# Autodesk Inventor assembly: 部件1
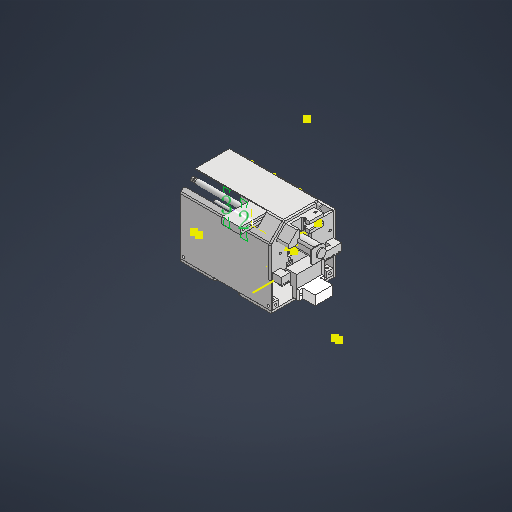
[picture p0: Inventor's stored thumbnail of the model, 512x512]
Saved by Autodesk Inventor 2025 (Build 290162000, 162)
## iProperties
Created: 2025-11-30
Part Number: 部件1
Document SubType Name: Assembly
Designer: XH
Author: XH
## Documents named in this file (41)
- C:\1A_Engineering_files\braille-printer-v2\3D文件\部件1.iam
- C:\1A_Engineering_files\braille-printer-v2\3D文件\便签.ipt
- C:\1A_Engineering_files\braille-printer-v2\3D文件\针头主体.iam
- C:\1A_Engineering_files\braille-printer-v2\3D文件\钢轴.ipt
- C:\1A_Engineering_files\braille-printer-v2\3D文件\阻挡X轴.ipt
- C:\Users\XH\Documents\Inventor\Content Center Files\R2025\zh-CN\AS 1420\AS 1420 - 1973 - M3 x 8.ipt
- C:\1A_Engineering_files\braille-printer-v2\3D文件\皮带.ipt
- C:\1A_Engineering_files\braille-printer-v2\3D文件\新配件\棍.ipt
- C:\1A_Engineering_files\braille-printer-v2\3D文件\电机.ipt
- C:\1A_Engineering_files\braille-printer-v2\3D文件\新配件\单轴.ipt
- C:\1A_Engineering_files\braille-printer-v2\3D文件\新配件\针头.iam
- C:\1A_Engineering_files\braille-printer-v2\3D文件\新配件\短轴3.ipt
- C:\1A_Engineering_files\braille-printer-v2\3D文件\新配件\连接件.ipt
- C:\1A_Engineering_files\braille-printer-v2\3D文件\阻挡X轴1.ipt
- C:\1A_Engineering_files\braille-printer-v2\3D文件\新配件\联轴器.ipt
- C:\1A_Engineering_files\braille-printer-v2\3D文件\新配件\外壳.ipt
- C:\1A_Engineering_files\braille-printer-v2\3D文件\新配件\大外壳.ipt
- C:\1A_Engineering_files\braille-printer-v2\3D文件\8D0A9F84C0C62D41F58A2185E0A23325.ipt
- C:\1A_Engineering_files\braille-printer-v2\3D文件\电机转接板.ipt
- C:\1A_Engineering_files\braille-printer-v2\3D文件\新配件\连接件电机.ipt
- C:\1A_Engineering_files\braille-printer-v2\3D文件\新配件\底板.ipt
- C:\1A_Engineering_files\braille-printer-v2\3D文件\新配件\底板2.ipt
- C:\1A_Engineering_files\braille-printer-v2\3D文件\新配件\8X.ipt
- C:\1A_Engineering_files\braille-printer-v2\3D文件\电池.ipt
- C:\1A_Engineering_files\braille-printer-v2\3D文件\ESP32.ipt
- C:\1A_Engineering_files\braille-printer-v2\3D文件\轴承3.7.3.ipt
- C:\1A_Engineering_files\braille-printer-v2\3D文件\入纸卡件.ipt
- C:\1A_Engineering_files\braille-printer-v2\3D文件\obj_2_1.齿条.STEP.ipt
- C:\1A_Engineering_files\braille-printer-v2\3D文件\obj_1_齿轮.STEP.ipt
- C:\1A_Engineering_files\braille-printer-v2\3D文件\Y轴杠轴.ipt
- C:\1A_Engineering_files\braille-printer-v2\3D文件\obj_3_外壳.STL.ipt
- C:\1A_Engineering_files\braille-printer-v2\3D文件\新配件\obj_2_1.齿条.STEP.ipt
- C:\1A_Engineering_files\braille-printer-v2\3D文件\obj_3_外1壳.STL.ipt
- C:\1A_Engineering_files\braille-printer-v2\3D文件\外宽挤压.ipt
- C:\1A_Engineering_files\braille-printer-v2\3D文件\小短轴.ipt
- C:\1A_Engineering_files\braille-printer-v2\3D文件\前轴固定.ipt
- C:\1A_Engineering_files\braille-printer-v2\3D文件\轴套.ipt
- C:\1A_Engineering_files\braille-printer-v2\3D文件\打印伸缩轴.ipt
- C:\1A_Engineering_files\braille-printer-v2\3D文件\铜套.ipt
- C:\1A_Engineering_files\braille-printer-v2\3D文件\新配件\滚纸.ipt
- C:\1A_Engineering_files\braille-printer-v2\3D文件\Z轴.ipt
## Components (66 placed, 39 different names)
1. 便签:1
2. 针头主体:1 [sub-assembly] — 配合:5, 配合:34, 表面齐平:19, 配合:198, 配合:199, 配合:200
3. 钢轴:2 — 配合:5, 表面齐平:14, 配合:83
4. 钢轴:3 — 配合:34, 表面齐平:14, 配合:75, 配合:76, 配合:82
5. AS 1420 - 公制 M3 x 8:1 — 配合:79, 配合:80
6. AS 1420 - 公制 M3 x 8:2 — 配合:77, 配合:78
7. 皮带:1
8. 棍:1 — 表面齐平:18, 配合:72
9. 棍:3 — 表面齐平:16, 配合:70
10. 棍:5 — 表面齐平:17, 配合:71
11. 电机:1 — 配合:73
12. 棍:6 — 表面齐平:18, 配合:68
13. 棍:7 — 表面齐平:16, 配合:69
14. 棍:8 — 表面齐平:17, 配合:67
15. 单轴:1
16. 针头:1 [sub-assembly] — 表面齐平:19, 配合:193, 配合:194, 配合:195, 配合:196, 配合:198, 配合:199, 配合:200
17. 短轴3:1 — 配合:67, 配合:68, 配合:69, 配合:201, 配合:204, 配合:211, 配合:214, 配合:288
18. 短轴3:2 — 配合:70, 配合:71, 配合:72, 配合:73, 配合:103, 配合:203, 表面齐平:29, 配合:212, 配合:289
19. 阻挡X轴:2 — 配合:75, 配合:76, 配合:77, 配合:78, 配合:79, 配合:80, 配合:100, 表面齐平:24, 表面齐平:25, 配合:210, 配合:213, 表面齐平:40, 配合:266, 配合:275, 配合:277, 配合:280
20. 连接件:1 — 配合:100, 配合:210, 配合:212, 配合:213, 配合:214
21. 阻挡X轴1:1 — 配合:82, 配合:83, 配合:104, 配合:105, 配合:123, 配合:221, 表面齐平:30, 表面齐平:31, 表面齐平:32, 配合:233, 表面齐平:33, 配合:234, 配合:278, 配合:293
22. 联轴器:1 — 配合:103
23. 外壳:1 — 配合:104
24. 大外壳:1 — 配合:105, 表面齐平:27, 配合:282, 配合:283, 配合:284
25. 电机转接板:1
26. 连接件电机:1 — 配合:123
27. 底板:1 — 表面齐平:24, 表面齐平:27, 配合:197, 表面齐平:28, 表面齐平:40, 配合:264, 表面齐平:43, 配合:275, 配合:281, 表面齐平:44, 配合:285, 配合:287
28. 底板2:1 — 表面齐平:25, 配合:232, 配合:234, 配合:265, 表面齐平:43, 配合:276, 配合:279, 配合:286, 表面齐平:45
29. 8X:2 — 配合:264, 配合:265, 配合:266
30. AS 1420 - 公制 M3 x 8:3 — 配合:193, 配合:194
31. AS 1420 - 公制 M3 x 8:4 — 配合:195, 配合:196
32. 电池:1
33. ESP32:1 — 配合:197, 表面齐平:28
34. 轴承3.7.3:1 — 配合:201, 配合:211
35. 轴承3.7.3:2 — 配合:203, 表面齐平:29
36. 轴承3.7.3:3 — 配合:204
37. 入纸卡件:1 — 配合:221, 表面齐平:30
38. obj_2_1.齿条.STEP:1 — 表面齐平:31, 表面齐平:32, 配合:233, 表面齐平:33, 配合:238, 配合:239
39. obj_1_齿轮.STEP:1 — 配合:229, 配合:231
40. 8D0A9F84C0C62D41F58A2185E0A23325:7 — 配合:229, 配合:231, 配合:236, 配合:237, 表面齐平:34, 配合:247
41. 8D0A9F84C0C62D41F58A2185E0A23325:8 — 配合:240, 配合:243, 表面齐平:36, 配合:244
42. Y轴杠轴:1 — 配合:232, 配合:260, 配合:290, 配合:294
43. 短轴3:3 — 配合:245, 配合:250, 配合:253
44. obj_3_外壳.STL:1 — 配合:236, 配合:237, 表面齐平:34, 配合:238, 配合:239, 表面齐平:37, 配合:270, 配合:271
45. obj_2_1.齿条.STEP:2 — 表面齐平:35, 配合:241, 配合:242, 配合:245
46. obj_1_齿轮.STEP:2 — 配合:240, 表面齐平:35
47. obj_3_外1壳.STL:1 — 配合:241, 配合:242, 配合:243, 表面齐平:36, 配合:244, 表面齐平:37, 配合:246, 配合:258, 配合:259
48. 外宽挤压:1 — 配合:246, 配合:247, 配合:258, 配合:259, 配合:260, 配合:270, 配合:271, 配合:272, 配合:274, 配合:295
49. 小短轴:1 — 配合:248, 配合:249, 配合:256
50. 前轴固定:1 — 配合:248, 配合:249, 配合:250
51. 前轴固定:2 — 配合:253, 配合:254, 配合:255
52. 小短轴:2 — 配合:254, 配合:255, 配合:257
53. 轴套:1 — 配合:256, 表面齐平:38, 表面齐平:39, 配合:267, 配合:268
54. 轴套:2 — 配合:257, 表面齐平:38, 表面齐平:39, 配合:269, 表面齐平:42
55. 打印伸缩轴:1 — 配合:267, 配合:268, 配合:272
56. 打印伸缩轴:2 — 配合:269, 表面齐平:42, 配合:274
57. 8X:6 — 配合:276, 配合:277
58. 8X:7 — 配合:278, 配合:279
59. 8X:8 — 配合:280, 配合:281, 配合:282, 配合:283
60. 8X:9 — 配合:284, 表面齐平:44, 配合:285
61. 8X:10 — 配合:286, 表面齐平:45, 配合:287
62. 轴套:3 — 配合:288, 表面齐平:46, 配合:291
63. 轴套:4 — 配合:289, 表面齐平:46, 表面齐平:47, 配合:292
64. 铜套:1 — 配合:290, 表面齐平:48
65. 滚纸:1 — 表面齐平:47, 配合:291, 配合:292, 配合:293
66. Z轴:1 — 配合:294, 表面齐平:48, 配合:295
## Relationships (126: Mate 98, Flush 28)
- 配合:5 [Mate]: 针头主体:1 ↔ 钢轴:2
- 配合:34 [Mate]: 针头主体:1 ↔ 钢轴:3
- 表面齐平:14 [Flush]: 钢轴:2 ↔ 钢轴:3
- 表面齐平:16 [Flush]: 棍:3 ↔ 棍:7
- 表面齐平:17 [Flush]: 棍:5 ↔ 棍:8
- 表面齐平:18 [Flush]: 棍:1 ↔ 棍:6
- 表面齐平:19 [Flush]: 针头主体:1 ↔ 针头:1
- 配合:67 [Mate]: 棍:8 ↔ 短轴3:1
- 配合:68 [Mate]: 棍:6 ↔ 短轴3:1
- 配合:69 [Mate]: 棍:7 ↔ 短轴3:1
- 配合:70 [Mate]: 棍:3 ↔ 短轴3:2
- 配合:71 [Mate]: 棍:5 ↔ 短轴3:2
- 配合:72 [Mate]: 棍:1 ↔ 短轴3:2
- 配合:73 [Mate]: 电机:1 ↔ 短轴3:2
- 配合:75 [Mate]: 钢轴:3 ↔ 阻挡X轴:2
- 配合:76 [Mate]: 钢轴:3 ↔ 阻挡X轴:2
- 配合:77 [Mate]: AS 1420 - 公制 M3 x 8:2 ↔ 阻挡X轴:2
- 配合:78 [Mate]: AS 1420 - 公制 M3 x 8:2 ↔ 阻挡X轴:2
- 配合:79 [Mate]: AS 1420 - 公制 M3 x 8:1 ↔ 阻挡X轴:2
- 配合:80 [Mate]: AS 1420 - 公制 M3 x 8:1 ↔ 阻挡X轴:2
- 配合:82 [Mate]: 钢轴:3 ↔ 阻挡X轴1:1
- 配合:83 [Mate]: 钢轴:2 ↔ 阻挡X轴1:1
- 配合:100 [Mate]: 阻挡X轴:2 ↔ 连接件:1
- 配合:103 [Mate]: 短轴3:2 ↔ 联轴器:1
- 配合:104 [Mate]: 阻挡X轴1:1 ↔ 外壳:1
- 配合:105 [Mate]: 阻挡X轴1:1 ↔ 大外壳:1
- 配合:123 [Mate]: 阻挡X轴1:1 ↔ 连接件电机:1
- 表面齐平:24 [Flush]: 阻挡X轴:2 ↔ 底板:1
- 表面齐平:25 [Flush]: 阻挡X轴:2 ↔ 底板2:1
- 表面齐平:27 [Flush]: 大外壳:1 ↔ 底板:1
- 配合:193 [Mate]: 针头:1 ↔ AS 1420 - 公制 M3 x 8:3
- 配合:194 [Mate]: 针头:1 ↔ AS 1420 - 公制 M3 x 8:3
- 配合:195 [Mate]: 针头:1 ↔ AS 1420 - 公制 M3 x 8:4
- 配合:196 [Mate]: 针头:1 ↔ AS 1420 - 公制 M3 x 8:4
- 配合:197 [Mate]: 底板:1 ↔ ESP32:1
- 表面齐平:28 [Flush]: 底板:1 ↔ ESP32:1
- 配合:198 [Mate]: 针头主体:1 ↔ 针头:1
- 配合:199 [Mate]: 针头主体:1 ↔ 针头:1
- 配合:200 [Mate]: 针头主体:1 ↔ 针头:1
- 配合:201 [Mate]: 短轴3:1 ↔ 轴承3.7.3:1
- 配合:203 [Mate]: 短轴3:2 ↔ 轴承3.7.3:2
- 表面齐平:29 [Flush]: 短轴3:2 ↔ 轴承3.7.3:2
- 配合:204 [Mate]: 短轴3:1 ↔ 轴承3.7.3:3
- 配合:210 [Mate]: 阻挡X轴:2 ↔ 连接件:1
- 配合:211 [Mate]: 短轴3:1 ↔ 轴承3.7.3:1
- 配合:212 [Mate]: 短轴3:2 ↔ 连接件:1
- 配合:213 [Mate]: 阻挡X轴:2 ↔ 连接件:1
- 配合:214 [Mate]: 短轴3:1 ↔ 连接件:1
- 配合:221 [Mate]: 阻挡X轴1:1 ↔ 入纸卡件:1
- 表面齐平:30 [Flush]: 阻挡X轴1:1 ↔ 入纸卡件:1
- 配合:229 [Mate]: obj_1_齿轮.STEP:1 ↔ 8D0A9F84C0C62D41F58A2185E0A23325:7
- 配合:231 [Mate]: obj_1_齿轮.STEP:1 ↔ 8D0A9F84C0C62D41F58A2185E0A23325:7
- 配合:232 [Mate]: 底板2:1 ↔ Y轴杠轴:1
- 表面齐平:31 [Flush]: 阻挡X轴1:1 ↔ obj_2_1.齿条.STEP:1
- 表面齐平:32 [Flush]: 阻挡X轴1:1 ↔ obj_2_1.齿条.STEP:1
- 配合:233 [Mate]: 阻挡X轴1:1 ↔ obj_2_1.齿条.STEP:1
- 表面齐平:33 [Flush]: 阻挡X轴1:1 ↔ obj_2_1.齿条.STEP:1
- 配合:234 [Mate]: 阻挡X轴1:1 ↔ 底板2:1
- 配合:236 [Mate]: 8D0A9F84C0C62D41F58A2185E0A23325:7 ↔ obj_3_外壳.STL:1
- 配合:237 [Mate]: 8D0A9F84C0C62D41F58A2185E0A23325:7 ↔ obj_3_外壳.STL:1
- 表面齐平:34 [Flush]: 8D0A9F84C0C62D41F58A2185E0A23325:7 ↔ obj_3_外壳.STL:1
- 配合:238 [Mate]: obj_2_1.齿条.STEP:1 ↔ obj_3_外壳.STL:1
- 配合:239 [Mate]: obj_2_1.齿条.STEP:1 ↔ obj_3_外壳.STL:1
- 配合:240 [Mate]: 8D0A9F84C0C62D41F58A2185E0A23325:8 ↔ obj_1_齿轮.STEP:2
- 表面齐平:35 [Flush]: obj_2_1.齿条.STEP:2 ↔ obj_1_齿轮.STEP:2
- 配合:241 [Mate]: obj_2_1.齿条.STEP:2 ↔ obj_3_外1壳.STL:1
- 配合:242 [Mate]: obj_2_1.齿条.STEP:2 ↔ obj_3_外1壳.STL:1
- 配合:243 [Mate]: 8D0A9F84C0C62D41F58A2185E0A23325:8 ↔ obj_3_外1壳.STL:1
- 表面齐平:36 [Flush]: 8D0A9F84C0C62D41F58A2185E0A23325:8 ↔ obj_3_外1壳.STL:1
- 配合:244 [Mate]: 8D0A9F84C0C62D41F58A2185E0A23325:8 ↔ obj_3_外1壳.STL:1
- 配合:245 [Mate]: 短轴3:3 ↔ obj_2_1.齿条.STEP:2
- 表面齐平:37 [Flush]: obj_3_外壳.STL:1 ↔ obj_3_外1壳.STL:1
- 配合:246 [Mate]: obj_3_外1壳.STL:1 ↔ 外宽挤压:1
- 配合:247 [Mate]: 8D0A9F84C0C62D41F58A2185E0A23325:7 ↔ 外宽挤压:1
- 配合:248 [Mate]: 小短轴:1 ↔ 前轴固定:1
- 配合:249 [Mate]: 小短轴:1 ↔ 前轴固定:1
- 配合:250 [Mate]: 短轴3:3 ↔ 前轴固定:1
- 配合:253 [Mate]: 短轴3:3 ↔ 前轴固定:2
- 配合:254 [Mate]: 前轴固定:2 ↔ 小短轴:2
- 配合:255 [Mate]: 前轴固定:2 ↔ 小短轴:2
- 配合:256 [Mate]: 小短轴:1 ↔ 轴套:1
- 配合:257 [Mate]: 小短轴:2 ↔ 轴套:2
- 表面齐平:38 [Flush]: 轴套:1 ↔ 轴套:2
- 配合:258 [Mate]: obj_3_外1壳.STL:1 ↔ 外宽挤压:1
- 配合:259 [Mate]: obj_3_外1壳.STL:1 ↔ 外宽挤压:1
- 配合:260 [Mate]: Y轴杠轴:1 ↔ 外宽挤压:1
- 表面齐平:39 [Flush]: 轴套:1 ↔ 轴套:2
- 表面齐平:40 [Flush]: 阻挡X轴:2 ↔ 底板:1
- 配合:264 [Mate]: 底板:1 ↔ 8X:2
- 配合:265 [Mate]: 底板2:1 ↔ 8X:2
- 配合:266 [Mate]: 阻挡X轴:2 ↔ 8X:2
- 配合:267 [Mate]: 轴套:1 ↔ 打印伸缩轴:1
- 配合:268 [Mate]: 轴套:1 ↔ 打印伸缩轴:1
- 配合:269 [Mate]: 轴套:2 ↔ 打印伸缩轴:2
- 配合:270 [Mate]: obj_3_外壳.STL:1 ↔ 外宽挤压:1
- 配合:271 [Mate]: obj_3_外壳.STL:1 ↔ 外宽挤压:1
- 表面齐平:42 [Flush]: 轴套:2 ↔ 打印伸缩轴:2
- 配合:272 [Mate]: 外宽挤压:1 ↔ 打印伸缩轴:1
- 配合:274 [Mate]: 外宽挤压:1 ↔ 打印伸缩轴:2
- 表面齐平:43 [Flush]: 底板:1 ↔ 底板2:1
- 配合:275 [Mate]: 阻挡X轴:2 ↔ 底板:1
- 配合:276 [Mate]: 底板2:1 ↔ 8X:6
- 配合:277 [Mate]: 阻挡X轴:2 ↔ 8X:6
- 配合:278 [Mate]: 阻挡X轴1:1 ↔ 8X:7
- 配合:279 [Mate]: 底板2:1 ↔ 8X:7
- 配合:280 [Mate]: 阻挡X轴:2 ↔ 8X:8
- 配合:281 [Mate]: 底板:1 ↔ 8X:8
- 配合:282 [Mate]: 大外壳:1 ↔ 8X:8
- 配合:283 [Mate]: 大外壳:1 ↔ 8X:8
- 配合:284 [Mate]: 大外壳:1 ↔ 8X:9
- 表面齐平:44 [Flush]: 底板:1 ↔ 8X:9
- 配合:285 [Mate]: 底板:1 ↔ 8X:9
- 配合:286 [Mate]: 底板2:1 ↔ 8X:10
- 表面齐平:45 [Flush]: 底板2:1 ↔ 8X:10
- 配合:287 [Mate]: 底板:1 ↔ 8X:10
- 配合:288 [Mate]: 短轴3:1 ↔ 轴套:3
- 配合:289 [Mate]: 短轴3:2 ↔ 轴套:4
- 表面齐平:46 [Flush]: 轴套:3 ↔ 轴套:4
- 配合:290 [Mate]: Y轴杠轴:1 ↔ 铜套:1
- 表面齐平:47 [Flush]: 轴套:4 ↔ 滚纸:1
- 配合:291 [Mate]: 轴套:3 ↔ 滚纸:1
- 配合:292 [Mate]: 轴套:4 ↔ 滚纸:1
- 配合:293 [Mate]: 阻挡X轴1:1 ↔ 滚纸:1
- 配合:294 [Mate]: Y轴杠轴:1 ↔ Z轴:1
- 表面齐平:48 [Flush]: 铜套:1 ↔ Z轴:1
- 配合:295 [Mate]: 外宽挤压:1 ↔ Z轴:1
